# Autodesk Inventor assembly: arm attachments SUB
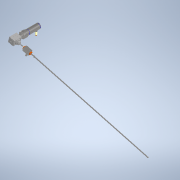
[picture p0: Inventor's stored thumbnail of the model, 180x180]
Saved by Autodesk Inventor 2021 (Build 250183000, 183)
## iProperties
Created: 2021-03-29
Part Number: arm attachments SUB
Document SubType Name: Assembly
Designer: Work
Author: Work
## Documents named in this file (7)
- C:\Users\Work\OneDrive - Brookhaven National Laboratory\Daniels, William intern HPR station\Arm\arm attachments SUB.iam
- C:\Users\Work\OneDrive - Brookhaven National Laboratory\Daniels, William intern HPR station\Arm\Z18936-A FULL ASSEMBLY.iam
- C:\Users\Work\OneDrive - Brookhaven National Laboratory\Daniels, William intern HPR station\Arm\AKMH23x-CCTNCAFK.ipt
- C:\Users\Work\OneDrive - Brookhaven National Laboratory\Daniels, William intern HPR station\Arm\AQT060-010-0-MMR-724.iam
- C:\Users\Work\OneDrive - Brookhaven National Laboratory\Daniels, William intern HPR station\Arm\HW-00-4.1-INT.ipt
- C:\Users\Work\OneDrive - Brookhaven National Laboratory\Daniels, William intern HPR station\Arm\wand.ipt
- C:\Users\Work\OneDrive - Brookhaven National Laboratory\Daniels, William intern HPR station\Arm\TD 010-CSTM.ipt
## Components (6 placed, 6 different names)
1. Z18936-A FULL ASSEMBLY:1 [sub-assembly] — Rotational:1, Rigid:3
2. AKMH23x-CCTNCAFK:1 — Rigid:1
3. AQT060-010-0-MMR-724:1 [sub-assembly] — Rigid:1, Rigid:2
4. HW-00-4.1-INT:1 — Rigid:2, Rotational:1
5. wand:1 — Rigid:3, Rigid:4
6. TD 010-CSTM:1 — Rigid:4
## Relationships (5: WeldJoint 4, RevoluteJoint 1)
- Rigid:1 [WeldJoint]: AKMH23x-CCTNCAFK:1 ↔ AQT060-010-0-MMR-724:1
- Rigid:2 [WeldJoint]: AQT060-010-0-MMR-724:1 ↔ HW-00-4.1-INT:1
- Rotational:1 [RevoluteJoint]: Z18936-A FULL ASSEMBLY:1 ↔ HW-00-4.1-INT:1
- Rigid:3 [WeldJoint]: Z18936-A FULL ASSEMBLY:1 ↔ wand:1
- Rigid:4 [WeldJoint]: wand:1 ↔ TD 010-CSTM:1
